# Autodesk Inventor assembly: belt fixture
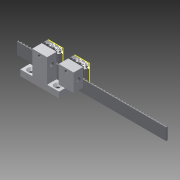
[picture p0: Inventor's stored thumbnail of the model, 180x180]
Saved by Autodesk Inventor 2015 SP1 (Build 190203100, 203)
## iProperties
Created: 2015-04-24
Part Number: belt fixture
Document SubType Name: Assembly
Designer: ubik
Author: ubik
## Documents named in this file (6)
- C:\Users\ubik\Dropbox\DueTech\cable test\belt fixture.iam
- C:\Users\ubik\Dropbox\DueTech\cable test\T2.5 belt.ipt
- C:\Users\ubik\Dropbox\DueTech\cable test\T2.5 belt holder.ipt
- C:\Users\ubik\Dropbox\DueTech\cable test\T2.5 belt\T2.5 belt-10.ipt
- C:\Users\ubik\Dropbox\DueTech\cable test\belt clamp.ipt
- C:\Users\ubik\Dropbox\DueTech\cable test\T2.5 belt holder fixed.ipt
## Components (5 placed, 4 different names)
1. T2.5 belt holder:1 — Flush:7, Flush:8
2. belt clamp:1 — Flush:5, Flush:6
3. belt clamp:2 — Flush:5, Flush:6, Flush:9
4. T2.5 belt holder fixed:1 — Flush:7, Flush:8, Flush:9, Mate:1
5. T2.5 belt-10:2 — Mate:1
## Relationships (6: Flush 5, Mate 1)
- Flush:5: belt clamp:1 ↔ belt clamp:2
- Flush:6: belt clamp:1 ↔ belt clamp:2
- Flush:7: T2.5 belt holder:1 ↔ T2.5 belt holder fixed:1
- Flush:8: T2.5 belt holder:1 ↔ T2.5 belt holder fixed:1
- Flush:9: belt clamp:2 ↔ T2.5 belt holder fixed:1
- Mate:1: T2.5 belt holder fixed:1 ↔ T2.5 belt-10:2
